# Autodesk Inventor assembly: grand desain
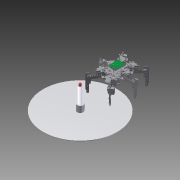
[picture p0: Inventor's stored thumbnail of the model, 180x180]
Saved by Autodesk Inventor 2012 (Build 160160000, 160)
## iProperties
Created: 2013-12-07
Part Number: grand desain
Document SubType Name: Assembly
Designer: Irwan Haryanto
Author: Irwan Haryanto
## Documents named in this file (10)
- D:\Revenant\robot baru 2014\grand desain.iam
- D:\Revenant\robot baru 2014\layer 2 + horn.iam
- D:\Revenant\robot baru 2014\coxa kiri.iam
- D:\Revenant\robot baru 2014\femur +horn.iam
- D:\Revenant\robot baru 2014\tibia kiri.iam
- D:\Revenant\robot baru 2014\coxa kanan.iam
- D:\Revenant\robot baru 2014\tibia kanan.iam
- D:\Revenant\robot baru 2014\layer 1.ipt
- D:\Revenant\robot baru 2014\spacer 5 cm.ipt
- D:\Revenant\robot baru 2014\lilin + dudukan + alas.ipt
## Components (25 placed, 9 different names)
1. layer 2 + horn:1 [sub-assembly] — Insert:1, Insert:2, Insert:3, Insert:19, Insert:20, Insert:21, Insert:24, Insert:25, Insert:26, Insert:27
2. coxa kiri:1 [sub-assembly] — Insert:1, Insert:6, Insert:22
3. coxa kiri:2 [sub-assembly] — Insert:3, Insert:4
4. coxa kiri:3 [sub-assembly] — Insert:2, Insert:5, Insert:23
5. femur +horn:1 [sub-assembly] — Insert:4, Insert:7
6. femur +horn:2 [sub-assembly] — Insert:5, Insert:8
7. femur +horn:3 [sub-assembly] — Insert:6, Insert:9
8. tibia kiri:1 [sub-assembly] — Insert:7
9. tibia kiri:2 [sub-assembly] — Insert:8
10. tibia kiri:3 [sub-assembly] — Insert:9
11. coxa kanan:1 [sub-assembly] — Insert:13, Insert:21
12. coxa kanan:2 [sub-assembly] — Insert:14, Insert:20
13. coxa kanan:3 [sub-assembly] — Insert:15, Insert:19
14. femur +horn:4 [sub-assembly] — Insert:13, Insert:16
15. femur +horn:5 [sub-assembly] — Insert:15, Insert:18
16. femur +horn:6 [sub-assembly] — Insert:14, Insert:17
17. tibia kanan:1 [sub-assembly] — Insert:16
18. tibia kanan:2 [sub-assembly] — Insert:17
19. tibia kanan:3 [sub-assembly] — Insert:18
20. layer 1:1 — Insert:22, Insert:23
21. spacer 5 cm:1 — Insert:24
22. spacer 5 cm:2 — Insert:25
23. spacer 5 cm:3 — Insert:26
24. spacer 5 cm:4 — Insert:27
25. lilin + dudukan + alas:1
## Relationships (24: Insert 24)
- Insert:1: layer 2 + horn:1 ↔ coxa kiri:1
- Insert:2: layer 2 + horn:1 ↔ coxa kiri:3
- Insert:3: layer 2 + horn:1 ↔ coxa kiri:2
- Insert:4: coxa kiri:2 ↔ femur +horn:1
- Insert:5: coxa kiri:3 ↔ femur +horn:2
- Insert:6: coxa kiri:1 ↔ femur +horn:3
- Insert:7: femur +horn:1 ↔ tibia kiri:1
- Insert:8: femur +horn:2 ↔ tibia kiri:2
- Insert:9: femur +horn:3 ↔ tibia kiri:3
- Insert:13: coxa kanan:1 ↔ femur +horn:4
- Insert:14: coxa kanan:2 ↔ femur +horn:6
- Insert:15: coxa kanan:3 ↔ femur +horn:5
- Insert:16: femur +horn:4 ↔ tibia kanan:1
- Insert:17: femur +horn:6 ↔ tibia kanan:2
- Insert:18: femur +horn:5 ↔ tibia kanan:3
- Insert:19: layer 2 + horn:1 ↔ coxa kanan:3
- Insert:20: layer 2 + horn:1 ↔ coxa kanan:2
- Insert:21: layer 2 + horn:1 ↔ coxa kanan:1
- Insert:22 (5 mm): coxa kiri:1 ↔ layer 1:1
- Insert:23: coxa kiri:3 ↔ layer 1:1
- Insert:24: layer 2 + horn:1 ↔ spacer 5 cm:1
- Insert:25: layer 2 + horn:1 ↔ spacer 5 cm:2
- Insert:26: layer 2 + horn:1 ↔ spacer 5 cm:3
- Insert:27: layer 2 + horn:1 ↔ spacer 5 cm:4
